# Autodesk Inventor assembly: valve assembly
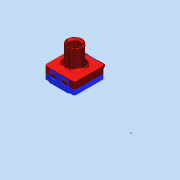
[picture p0: Inventor's stored thumbnail of the model, 180x180]
Saved by Autodesk Inventor 2020 (Build 240168000, 168)
## iProperties
Created: 2020-04-08
Part Number: valve assembly
Document SubType Name: Assembly
Designer: Simon
Author: Simon
## Documents named in this file (3)
- D:\GrabCAD\MTL Ventilator Design\Filter housing with o ring\valve assembly.iam
- D:\GrabCAD\MTL Ventilator Design\Filter housing with o ring\check valve v2 v1.ipt
- D:\GrabCAD\MTL Ventilator Design\Filter housing with o ring\filter_connector v1 (1).ipt
## Components (2 placed, 2 different names)
1. check valve v2 v1:1 — Mate:1, Flush:1
2. filter_connector v1 (1):1 — Mate:1, Flush:1
## Relationships (2: Mate 1, Flush 1)
- Mate:1: check valve v2 v1:1 ↔ filter_connector v1 (1):1
- Flush:1: check valve v2 v1:1 ↔ filter_connector v1 (1):1
